# Autodesk Inventor assembly: MotorMount
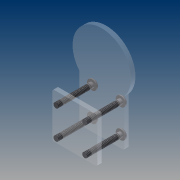
[picture p0: Inventor's stored thumbnail of the model, 180x180]
Saved by Autodesk Inventor 2011 SP1 (Build 150282100, 282)
## iProperties
Created: 2011-07-18
Part Number: MotorMount
Document SubType Name: Assembly
Designer: Nathan
Author: Nathan
## Documents named in this file (4)
- C:\Users\Nathan\Documents\Inventor\Quadcopter\MotorMount.iam
- C:\Users\Nathan\Documents\Inventor\Quadcopter\MotorMountTop.ipt
- C:\Users\Nathan\Documents\Inventor\Content Center Files\R2011\en-US\ANSI B18.6.3(26)\ANSI B18.6.3 - 6-32 UNC - 1(7).ipt
- C:\Users\Nathan\Documents\Inventor\Quadcopter\MotorMountBottom.ipt
## Components (6 placed, 3 different names)
1. MotorMountTop:1 — Mate:1, Mate:2, Mate:3, Mate:4, Mate:7, Mate:8, Mate:9, Mate:10, Mate:11
2. Cross Recessed Pan Head Machine Screw - Type II - Inch No. 6 - 32 - 1:1 — Mate:1, Mate:8
3. Cross Recessed Pan Head Machine Screw - Type II - Inch No. 6 - 32 - 1:2 — Mate:2, Mate:9
4. Cross Recessed Pan Head Machine Screw - Type II - Inch No. 6 - 32 - 1:3 — Mate:3, Mate:6, Mate:11
5. MotorMountBottom:1 — Mate:5, Mate:6, Mate:7
6. Cross Recessed Pan Head Machine Screw - Type II - Inch No. 6 - 32 - 1:4 — Mate:4, Mate:5, Mate:10
## Relationships (11: Mate 11)
- Mate:1: MotorMountTop:1 ↔ Cross Recessed Pan Head Machine Screw - Type II - Inch No. 6 - 32 - 1:1
- Mate:2: MotorMountTop:1 ↔ Cross Recessed Pan Head Machine Screw - Type II - Inch No. 6 - 32 - 1:2
- Mate:3: MotorMountTop:1 ↔ Cross Recessed Pan Head Machine Screw - Type II - Inch No. 6 - 32 - 1:3
- Mate:4: MotorMountTop:1 ↔ Cross Recessed Pan Head Machine Screw - Type II - Inch No. 6 - 32 - 1:4
- Mate:5: MotorMountBottom:1 ↔ Cross Recessed Pan Head Machine Screw - Type II - Inch No. 6 - 32 - 1:4
- Mate:6: Cross Recessed Pan Head Machine Screw - Type II - Inch No. 6 - 32 - 1:3 ↔ MotorMountBottom:1
- Mate:7 (15.875 mm): MotorMountTop:1 ↔ MotorMountBottom:1
- Mate:8: MotorMountTop:1 ↔ Cross Recessed Pan Head Machine Screw - Type II - Inch No. 6 - 32 - 1:1
- Mate:9: MotorMountTop:1 ↔ Cross Recessed Pan Head Machine Screw - Type II - Inch No. 6 - 32 - 1:2
- Mate:10: MotorMountTop:1 ↔ Cross Recessed Pan Head Machine Screw - Type II - Inch No. 6 - 32 - 1:4
- Mate:11: MotorMountTop:1 ↔ Cross Recessed Pan Head Machine Screw - Type II - Inch No. 6 - 32 - 1:3
